# Autodesk Inventor assembly: Ember
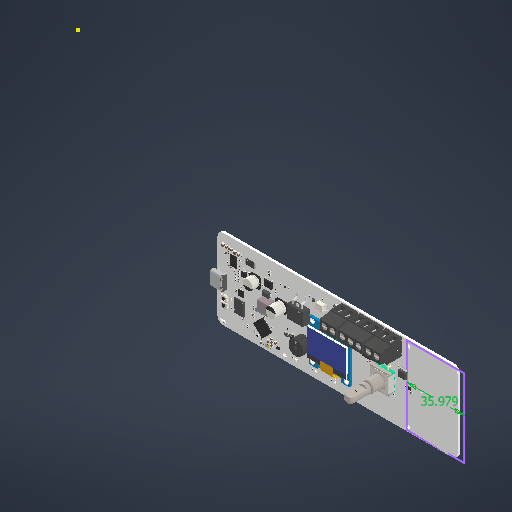
[picture p0: Inventor's stored thumbnail of the model, 512x512]
Saved by Autodesk Inventor 2026.1 (Build 301233020, 233B)
## iProperties
Created: 2025-11-22
Part Number: Ember
Document SubType Name: Assembly
Designer: Nathan
Author: Nathan
## Documents named in this file (3)
- C:\Users\Nathan\Documents\GitHub\ember\hardware\case\Ember.iam
- C:\Users\Nathan\Documents\GitHub\ember\hardware\board\ember\ember\ember.ipt
- C:\Users\Nathan\Documents\GitHub\ember\hardware\case\bottom_case.ipt
## Components (2 placed, 2 different names)
1. ember:1 — Flush:1
2. bottom_case:1 — Flush:1
## Relationships (1: Flush 1)
- Flush:1: ember:1 ↔ bottom_case:1
## Named parameters: CASE_WIDTH = 60 mm, CASE_LENGTH = 160 mm, BOTTOM_THICKNESS = 5 mm, TOP_THICKNESS = 5 mm
